# Autodesk Inventor assembly: 2017 Plate with 2018 boxes
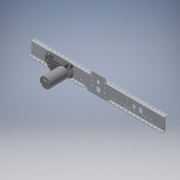
[picture p0: Inventor's stored thumbnail of the model, 180x180]
Saved by Autodesk Inventor 2018 (Build 220112000, 112)
## iProperties
Created: 2018-01-16
Part Number: 2017 Plate with 2018 boxes
Document SubType Name: Assembly
Designer: Apple
Author: Apple
## Documents named in this file (4)
- C:\Users\Apple\Documents\Inventor\2018 PowerUp\2017 Plate with 2018 boxes.iam
- C:\Users\Apple\Downloads\am-2952a_AM14U3_Inside_Plate.ipt
- C:\Users\Apple\Documents\Inventor\2018 PowerUp\AndyMark\Molded Assembly Rev 7 with am-0153 shaft_Long Micro Shaft.iam
- C:\Users\Apple\Documents\Inventor\2018 PowerUp\CIM motor-1.ipt
## Components (5 placed, 3 different names)
1. am-2952a_AM14U3_Inside_Plate:1 — Mate:3, Mate:4, Mate:7, Mate:8
2. Molded Assembly Rev 7 with am-0153 shaft_Long Micro Shaft:1 [sub-assembly] — Mate:3, Mate:4, Flush:1
3. CIM motor-1:1
4. Molded Assembly Rev 7 with am-0153 shaft_Long Micro Shaft:2 [sub-assembly] — Mate:7, Mate:8, Flush:1
5. CIM motor-1:2
## Relationships (9: Mate 8, Flush 1)
- [Mate]: Molded Assembly Rev 7 with am-0153 shaft_Long Micro Shaft:1 ↔ CIM motor-1:1
- [Mate]: Molded Assembly Rev 7 with am-0153 shaft_Long Micro Shaft:1 ↔ CIM motor-1:1
- Mate:3: am-2952a_AM14U3_Inside_Plate:1 ↔ Molded Assembly Rev 7 with am-0153 shaft_Long Micro Shaft:1
- Mate:4: am-2952a_AM14U3_Inside_Plate:1 ↔ Molded Assembly Rev 7 with am-0153 shaft_Long Micro Shaft:1
- [Mate]: Molded Assembly Rev 7 with am-0153 shaft_Long Micro Shaft:2 ↔ CIM motor-1:2
- [Mate]: Molded Assembly Rev 7 with am-0153 shaft_Long Micro Shaft:2 ↔ CIM motor-1:2
- Mate:7: am-2952a_AM14U3_Inside_Plate:1 ↔ Molded Assembly Rev 7 with am-0153 shaft_Long Micro Shaft:2
- Mate:8: am-2952a_AM14U3_Inside_Plate:1 ↔ Molded Assembly Rev 7 with am-0153 shaft_Long Micro Shaft:2
- Flush:1: Molded Assembly Rev 7 with am-0153 shaft_Long Micro Shaft:1 ↔ Molded Assembly Rev 7 with am-0153 shaft_Long Micro Shaft:2
## Named parameters: d5_d3 = 0 mm, d6_d10 = 0 mm
